# Autodesk Inventor assembly: Full Assembly V1
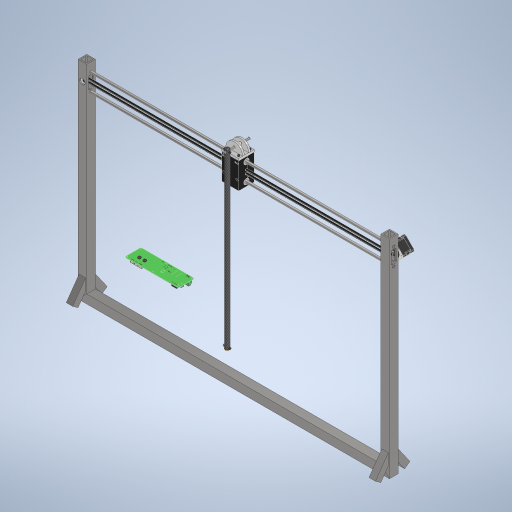
[picture p0: Inventor's stored thumbnail of the model, 512x512]
Saved by Autodesk Inventor 2023 (Build 270158000, 158)
## iProperties
Created: 2023-02-13
Part Number: Full Assembly V1
Document SubType Name: Assembly
Designer: mbear
Mass: 3026.54 g
Surface Area: 6379.54 cm^2
Volume: 1029.05 cm^3
Density: 2.9411 g/cm^3
Author: mbear
## Documents named in this file (21)
- C:\Users\mbear\OneDrive\Documents\Inventor\Inverted Pendulum\Full Assembly V1.iam
- C:\Users\mbear\OneDrive\Documents\Inventor\Inverted Pendulum\NEMA17 Model.ipt
- C:\Users\mbear\OneDrive\Documents\Inventor\Inverted Pendulum\Pendulum Tubing.ipt
- C:\Users\mbear\OneDrive\Documents\Inventor\Inverted Pendulum\Linear Rod.ipt
- C:\Users\mbear\OneDrive\Documents\Inventor\Inverted Pendulum\Carriage Axle V1.ipt
- C:\Users\mbear\OneDrive\Documents\Inventor\Inverted Pendulum\M3 Square Nut.ipt
- C:\Users\mbear\OneDrive\Documents\Inventor\Inverted Pendulum\Hex_Socket_M3x16.ipt
- C:\Users\mbear\OneDrive\Documents\Inventor\Inverted Pendulum\M3 Nyloc Nut.ipt
- C:\Users\mbear\OneDrive\Documents\Inventor\Inverted Pendulum\Brass Endweight.ipt
- C:\Users\mbear\OneDrive\Documents\Inventor\Inverted Pendulum\PendulumControllerBoard.iam
- C:\Users\mbear\OneDrive\Documents\Inventor\Inverted Pendulum\3764N101_High-Strength Gt Timing Belt Pulley.ipt
- C:\Users\mbear\OneDrive\Documents\Inventor\Inverted Pendulum\Carriage Belt.ipt
- C:\Users\mbear\OneDrive\Documents\Inventor\Inverted Pendulum\FrameAssembly V2.iam
- C:\Users\mbear\OneDrive\Documents\Inventor\Inverted Pendulum\Hex_Socket_M5x20.ipt
- C:\Users\mbear\OneDrive\Documents\Inventor\Inverted Pendulum\M5 Nyloc Nut.ipt
- C:\Users\mbear\OneDrive\Documents\Inventor\Inverted Pendulum\Carriage Top.ipt
- C:\Users\mbear\OneDrive\Documents\Inventor\Inverted Pendulum\Carriage Design Right.ipt
- C:\Users\mbear\OneDrive\Documents\Inventor\Inverted Pendulum\Carriage Design Left.ipt
- C:\Users\mbear\OneDrive\Documents\Inventor\Inverted Pendulum\Dry Bearing.ipt
- C:\Users\mbear\OneDrive\Documents\Inventor\Inverted Pendulum\Hex_Socket_M3x14.ipt
- C:\Users\mbear\OneDrive\Documents\Inventor\Inverted Pendulum\Carriage Axle Set Screw Holder.ipt
## Components (36 placed, 20 different names)
1. NEMA17 Model:1 — Insert:16, Insert:19, Insert:20
2. Linear Rod:1 — Mate:9, Mate:10, Insert:27
3. Linear Rod:2 — Insert:18, Insert:28, Mate:11
4. Carriage Axle V1:1 — Mate:3, Mate:4, Mate:14, Mate:15
5. Pendulum Tubing:1 — Mate:3, Mate:4, Mate:5, Flush:1, Mate:6, Mate:7, Mate:8
6. M3 Square Nut:1
7. M3 Square Nut:2
8. Hex_Socket_M3x16:1
9. Hex_Socket_M3x16:2
10. Hex_Socket_M3x16:3
11. Hex_Socket_M3x16:4
12. Hex_Socket_M3x16:5 — Mate:5, Insert:14, Flush:2
13. M3 Nyloc Nut:1 — Insert:14
14. Brass Endweight:1 — Mate:6, Mate:7
15. Hex_Socket_M3x16:6 — Mate:8, Flush:3, Insert:15
16. M3 Nyloc Nut:2 — Insert:15
17. PendulumControllerBoard:1 [sub-assembly]
18. 3764N101_High-Strength Gt Timing Belt Pulley:1 — Insert:16, Insert:17
19. Carriage Belt:1 — Insert:17, Angle:7
20. FrameAssembly V2:1 [sub-assembly] — Mate:9, Insert:18, Insert:19, Insert:20, Insert:21, Insert:22, Angle:7, Insert:27, Insert:28
21. Hex_Socket_M5x20:1 — Insert:21
22. M5 Nyloc Nut:1 — Insert:22
23. Carriage Top:1 — Mate:13, Flush:6, Flush:7, Mate:14, Insert:35
24. Carriage Design Right:1 — Mate:12, Flush:4, Flush:5, Insert:29, Insert:30, Angle:8, Angle:9, Insert:33, Insert:34
25. Carriage Design Left:1 — Insert:23, Insert:24, Insert:25, Insert:26, Mate:12, Flush:4, Flush:5, Mate:13, Flush:6, Flush:7, Insert:31, Insert:32, Angle:10, Angle:11
26. M3 Square Nut:3 — Insert:29, Angle:8
27. M3 Square Nut:4 — Insert:30, Angle:9
28. Dry Bearing:1 — Insert:24, Mate:11
29. Dry Bearing:2 — Insert:25
30. Dry Bearing:3 — Insert:23, Mate:10
31. Dry Bearing:4 — Insert:26
32. Hex_Socket_M3x14:1 — Insert:31
33. Hex_Socket_M3x14:2 — Insert:32
34. M3 Square Nut:5 — Insert:33, Angle:10
35. M3 Square Nut:6 — Insert:34, Angle:11
36. Carriage Axle Set Screw Holder:1 — Insert:35, Mate:15
## Relationships (47: Insert 22, Mate 13, Flush 7, Angle 5)
- Mate:3: Carriage Axle V1:1 ↔ Pendulum Tubing:1
- Mate:4: Carriage Axle V1:1 ↔ Pendulum Tubing:1
- Mate:5: Pendulum Tubing:1 ↔ Hex_Socket_M3x16:5
- Insert:14 (0.762 mm): Hex_Socket_M3x16:5 ↔ M3 Nyloc Nut:1
- Flush:1 (-6.35 mm): Pendulum Tubing:1
- Flush:2: Hex_Socket_M3x16:5
- Mate:6: Pendulum Tubing:1 ↔ Brass Endweight:1
- Mate:7: Pendulum Tubing:1 ↔ Brass Endweight:1
- Mate:8: Pendulum Tubing:1 ↔ Hex_Socket_M3x16:6
- Flush:3: Hex_Socket_M3x16:6
- Insert:15 (0.508 mm): Hex_Socket_M3x16:6 ↔ M3 Nyloc Nut:2
- Insert:16 (1.27 mm): NEMA17 Model:1 ↔ 3764N101_High-Strength Gt Timing Belt Pulley:1
- Insert:17 (0.7366 mm): 3764N101_High-Strength Gt Timing Belt Pulley:1 ↔ Carriage Belt:1
- Mate:9: Linear Rod:1 ↔ FrameAssembly V2:1
- Insert:18: Linear Rod:2 ↔ FrameAssembly V2:1
- Insert:19: NEMA17 Model:1 ↔ FrameAssembly V2:1
- Insert:20: NEMA17 Model:1 ↔ FrameAssembly V2:1
- Insert:21: FrameAssembly V2:1 ↔ Hex_Socket_M5x20:1
- Insert:22: FrameAssembly V2:1 ↔ M5 Nyloc Nut:1
- Angle:7 (0 deg): Carriage Belt:1 ↔ FrameAssembly V2:1
- Insert:23: Carriage Design Left:1 ↔ Dry Bearing:3
- Insert:24: Carriage Design Left:1 ↔ Dry Bearing:1
- Insert:25: Carriage Design Left:1 ↔ Dry Bearing:2
- Insert:26: Carriage Design Left:1 ↔ Dry Bearing:4
- Mate:10: Linear Rod:1 ↔ Dry Bearing:3
- Insert:27: Linear Rod:1 ↔ FrameAssembly V2:1
- Insert:28: Linear Rod:2 ↔ FrameAssembly V2:1
- Mate:11: Linear Rod:2 ↔ Dry Bearing:1
- Mate:12: Carriage Design Right:1 ↔ Carriage Design Left:1
- Flush:4: Carriage Design Right:1 ↔ Carriage Design Left:1
- Flush:5: Carriage Design Right:1 ↔ Carriage Design Left:1
- Mate:13: Carriage Top:1 ↔ Carriage Design Left:1
- Flush:6: Carriage Top:1 ↔ Carriage Design Left:1
- Flush:7: Carriage Top:1 ↔ Carriage Design Left:1
- Mate:14: Carriage Axle V1:1 ↔ Carriage Top:1
- Insert:29: Carriage Design Right:1 ↔ M3 Square Nut:3
- Insert:30: Carriage Design Right:1 ↔ M3 Square Nut:4
- Angle:8 (0 deg): Carriage Design Right:1 ↔ M3 Square Nut:3
- Angle:9 (0 deg): Carriage Design Right:1 ↔ M3 Square Nut:4
- Insert:31: Carriage Design Left:1 ↔ Hex_Socket_M3x14:1
- Insert:32: Carriage Design Left:1 ↔ Hex_Socket_M3x14:2
- Insert:33: Carriage Design Right:1 ↔ M3 Square Nut:5
- Angle:10 (0 deg): Carriage Design Left:1 ↔ M3 Square Nut:5
- Insert:34: Carriage Design Right:1 ↔ M3 Square Nut:6
- Angle:11 (0 deg): Carriage Design Left:1 ↔ M3 Square Nut:6
- Insert:35: Carriage Top:1 ↔ Carriage Axle Set Screw Holder:1
- Mate:15: Carriage Axle V1:1 ↔ Carriage Axle Set Screw Holder:1
